# Autodesk Inventor assembly: panel_waveguide
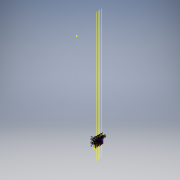
[picture p0: Inventor's stored thumbnail of the model, 180x180]
Saved by Autodesk Inventor 2017 (Build 210142000, 142)
## iProperties
Created: 2017-07-06
Part Number: panel_waveguide
Document SubType Name: Assembly
Designer: Zara
Author: Zara
## Documents named in this file (3)
- C:\Users\Zara\Documents\hera-cad\Node\Concept-ICTS\ICTS-20170411\panel_waveguide.iam
- C:\Users\Zara\Documents\hera-cad\Node\Concept-ICTS\ICTS-20170411\RD-A001-P001-REV0-cutouts.ipt
- C:\Users\Zara\Documents\hera-cad\Node\Concept-ICTS\ICTS-20170411\waveguide.ipt
## Components (5 placed, 2 different names)
1. RD-A001-P001-REV0-cutouts:1 — Mate:1, Angle:1, Mate:2, Angle:2, Mate:3, Angle:3, Mate:4, Angle:4, Mate:5, Mate:6, Mate:7, Mate:8
2. waveguide:1 — Mate:1, Angle:1, Mate:5
3. waveguide:2 — Mate:4, Angle:4, Mate:8
4. waveguide:3 — Mate:2, Angle:2, Mate:6
5. waveguide:4 — Mate:3, Angle:3, Mate:7
## Relationships (12: Mate 8, Angle 4)
- Mate:1: RD-A001-P001-REV0-cutouts:1 ↔ waveguide:1
- Angle:1 (0 deg): RD-A001-P001-REV0-cutouts:1 ↔ waveguide:1
- Mate:2: RD-A001-P001-REV0-cutouts:1 ↔ waveguide:3
- Angle:2 (0 deg): RD-A001-P001-REV0-cutouts:1 ↔ waveguide:3
- Mate:3: RD-A001-P001-REV0-cutouts:1 ↔ waveguide:4
- Angle:3 (0 deg): RD-A001-P001-REV0-cutouts:1 ↔ waveguide:4
- Mate:4: RD-A001-P001-REV0-cutouts:1 ↔ waveguide:2
- Angle:4 (0 deg): RD-A001-P001-REV0-cutouts:1 ↔ waveguide:2
- Mate:5: RD-A001-P001-REV0-cutouts:1 ↔ waveguide:1
- Mate:6: RD-A001-P001-REV0-cutouts:1 ↔ waveguide:3
- Mate:7: RD-A001-P001-REV0-cutouts:1 ↔ waveguide:4
- Mate:8: RD-A001-P001-REV0-cutouts:1 ↔ waveguide:2
